# Autodesk Inventor assembly: A1-19037-200-00 30in lateral
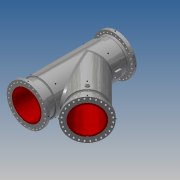
[picture p0: Inventor's stored thumbnail of the model, 180x180]
Saved by Autodesk Inventor 2017.3 (Build 213257000, 257)
## iProperties
Created: 2019-08-22
Part Number: A1-19037-200-00 30in lateral
Document SubType Name: Weldment
Designer: GVD
Project: A1-19037--CNUL Albian CST laterals
Weld Material: Steel, Mild, Welded
Mass: 6.1789e+06 g
Surface Area: 437297 cm^2
Volume: 814103 cm^3
Density: 7.58982 g/cm^3
Constructed By: Graeme_Van_Dongen
Project Name: CST laterals
Author: GVD
## Documents named in this file (15)
- C:\156Vault\A1 - Projects\A1-19\A1-19037--CNUL Albian CST laterals\A1-19037-200-00 30in lateral.iam
- N:\Inventor\Content Center Files\R2017\en-US\ANSI B18.3(08)\ANSI B18.3 - 1_2-13 UNC - 0.5(24).ipt
- N:\Inventor\Content Center Files\R2017\en-US\ASME B16.11(23)\ASME B16.11 Hex Head Plug 1_2.ipt
- N:\Inventor\Content Center Files\R2017\en-US\ASME B16.11(23)\ASME B16.11 Hex Head Plug 3_4.ipt
- N:\Inventor\Content Center Files\R2017\en-US\ASME B16.11(23)\ASME B16.11 Hex Head Plug 2.ipt
- C:\156Vault\A1 - Projects\A1-19\A1-19037--CNUL Albian CST laterals\A1-19037-200-04 30in CL300 RF flange - custom.ipt
- C:\156Vault\A1 - Projects\A1-19\A1-19037--CNUL Albian CST laterals\A1-19037-200-03 34in pipe.ipt
- C:\156Vault\A1 - Projects\A1-19\A1-19037--CNUL Albian CST laterals\A1-19037-200-01 Trunk shell.ipt
- C:\156Vault\A1 - Projects\A1-19\A1-19037--CNUL Albian CST laterals\A1-19037-200-02 Branch shell.ipt
- C:\156Vault\A1 - Projects\A1-19\A1-19037--CNUL Albian CST laterals\A1-19037-200-05 HCWI lateral.ipt
- C:\156Vault\A1 - Projects\A1-19\A1-19037--CNUL Albian CST laterals\A1-19037-200-06 HCWI liner - pup.ipt
- C:\156Vault\A1 - Projects\A1-19\A1-19037--CNUL Albian CST laterals\A1-19037-200-07 Trap rod.ipt
- C:\156Vault\A1 - Projects\A1-19\A1-19037--CNUL Albian CST laterals\A1-19037-200-08 2in x 38in threadolet.ipt
- C:\156Vault\A1 - Projects\Penticton Foundry\Tag mount - 6in.ipt
- C:\156Vault\A1 - Projects\A1-19\A1-19037--CNUL Albian CST laterals\A1-19037-200-03 34in pipe - flange assy.iam
## Components (61 placed, 14 different names)
1. A1-19037-200-04 30in CL300 RF flange - custom:2 — Insert:5, Insert:8, Mate:5, Angle:13, Angle:14, Mate:6, Mate:11, Angle:18, Mate:16, Angle:22, Tangent:5, Angle:23
2. A1-19037-200-04 30in CL300 RF flange - custom:3 — Insert:6, Insert:9, Mate:7, Angle:15, Angle:16, Mate:8, Mate:13, Angle:19, Mate:17, Angle:24, Tangent:6, Angle:25
3. A1-19037-200-05 HCWI lateral:1 — Insert:2, Angle:3, Insert:3, Angle:4, Insert:4, Angle:5, Flush:1, Mate:18, Angle:26
4. A1-19037-200-06 HCWI liner - pup:1 — Insert:2, Angle:3, Tangent:1
5. A1-19037-200-06 HCWI liner - pup:2 — Insert:3, Angle:4, Insert:5, Tangent:2
6. A1-19037-200-06 HCWI liner - pup:3 — Insert:4, Angle:5, Insert:6, Tangent:3
7. A1-19037-200-03 34in pipe:2 — Insert:8
8. A1-19037-200-03 34in pipe:3 — Insert:9
9. A1-19037-200-01 Trunk shell:1 — Flush:1, Mate:18, Angle:26, Flush:2, Mate:19, Angle:27, Mate:20, Angle:28, Tangent:7, Angle:29, Mate:21, Angle:30, Tangent:8, Angle:31, Mate:22, Angle:32, Tangent:9, Angle:33, Mate:23, Angle:34, Tangent:10, Angle:35, Tangent:12
10. A1-19037-200-02 Branch shell:1 — Flush:2, Mate:19, Angle:27, Mate:24, Mate:25, Angle:36, Mate:26, Angle:38, Tangent:11, Angle:39
11. ASME B16.11 Hex Head Plug 2:1 — Insert:10, Angle:37
12. A1-19037-200-08 2in x 38in threadolet:1 — Mate:24, Mate:25, Angle:36, Insert:10, Angle:37
13. A1-19037-200-03 34in pipe - flange assy:1 [sub-assembly]
14. A1-19037-200-07 Trap rod:1 — Tangent:1, Mate:10
15. Hexagon Socket Set Screw - Flat Point - Inch 1/2-13 UNC x 0.5:1 — Mate:10
16. ASME B16.11 Hex Head Plug 1/2:1
17. A1-19037-200-07 Trap rod:4
18. Hexagon Socket Set Screw - Flat Point - Inch 1/2-13 UNC x 0.5:4
19. ASME B16.11 Hex Head Plug 1/2:4
20. A1-19037-200-07 Trap rod:5
21. Hexagon Socket Set Screw - Flat Point - Inch 1/2-13 UNC x 0.5:5
22. ASME B16.11 Hex Head Plug 1/2:5
23. A1-19037-200-07 Trap rod:6
24. Hexagon Socket Set Screw - Flat Point - Inch 1/2-13 UNC x 0.5:6
25. ASME B16.11 Hex Head Plug 1/2:6
26. A1-19037-200-07 Trap rod:2 — Mate:5, Angle:13, Angle:14, Mate:6, Tangent:2, Mate:12
27. Hexagon Socket Set Screw - Flat Point - Inch 1/2-13 UNC x 0.5:2 — Mate:11, Mate:12, Angle:18
28. ASME B16.11 Hex Head Plug 1/2:2 — Mate:16, Angle:22, Tangent:5, Angle:23
29. A1-19037-200-07 Trap rod:7
30. Hexagon Socket Set Screw - Flat Point - Inch 1/2-13 UNC x 0.5:7
31. ASME B16.11 Hex Head Plug 1/2:7
32. A1-19037-200-07 Trap rod:8
33. Hexagon Socket Set Screw - Flat Point - Inch 1/2-13 UNC x 0.5:8
34. ASME B16.11 Hex Head Plug 1/2:8
35. A1-19037-200-07 Trap rod:9
36. Hexagon Socket Set Screw - Flat Point - Inch 1/2-13 UNC x 0.5:9
37. ASME B16.11 Hex Head Plug 1/2:9
38. A1-19037-200-07 Trap rod:3 — Mate:7, Angle:15, Angle:16, Mate:8, Tangent:3, Mate:14
39. Hexagon Socket Set Screw - Flat Point - Inch 1/2-13 UNC x 0.5:3 — Mate:13, Mate:14, Angle:19
40. ASME B16.11 Hex Head Plug 1/2:3 — Mate:17, Angle:24, Tangent:6, Angle:25
41. A1-19037-200-07 Trap rod:10
42. Hexagon Socket Set Screw - Flat Point - Inch 1/2-13 UNC x 0.5:10
43. ASME B16.11 Hex Head Plug 1/2:10
44. A1-19037-200-07 Trap rod:11
45. Hexagon Socket Set Screw - Flat Point - Inch 1/2-13 UNC x 0.5:11
46. ASME B16.11 Hex Head Plug 1/2:11
47. A1-19037-200-07 Trap rod:12
48. Hexagon Socket Set Screw - Flat Point - Inch 1/2-13 UNC x 0.5:12
49. ASME B16.11 Hex Head Plug 1/2:12
50. ASME B16.11 Hex Head Plug 3/4:1 — Mate:20, Angle:28, Tangent:7, Angle:29
51. ASME B16.11 Hex Head Plug 3/4:2 — Mate:21, Angle:30, Tangent:8, Angle:31
52. ASME B16.11 Hex Head Plug 3/4:3 — Mate:22, Angle:32, Tangent:9, Angle:33
53. ASME B16.11 Hex Head Plug 3/4:4 — Mate:23, Angle:34, Tangent:10, Angle:35
54. ASME B16.11 Hex Head Plug 3/4:5
55. ASME B16.11 Hex Head Plug 3/4:6
56. ASME B16.11 Hex Head Plug 3/4:7
57. ASME B16.11 Hex Head Plug 3/4:8
58. ASME B16.11 Hex Head Plug 3/4:9 — Mate:26, Angle:38, Tangent:11, Angle:39
59. ASME B16.11 Hex Head Plug 3/4:10
60. Tag mount - 6in:1 — Tangent:12
61. Tag mount - 6in:2
## Component patterns: (4 elements, first: A1-19037-200-07 Trap rod:1 + Hexagon Socket Set Screw - Flat Point - Inch 1/2-13 UNC x 0.5:1 + ASME B16.11 Hex Head Plug 1/2:1), (4 elements, first: A1-19037-200-07 Trap rod:2 + Hexagon Socket Set Screw - Flat Point - Inch 1/2-13 UNC x 0.5:2 + ASME B16.11 Hex Head Plug 1/2:2), (4 elements, first: A1-19037-200-07 Trap rod:3 + Hexagon Socket Set Screw - Flat Point - Inch 1/2-13 UNC x 0.5:3 + ASME B16.11 Hex Head Plug 1/2:3), (2 elements, first: ASME B16.11 Hex Head Plug 3/4:1 + ASME B16.11 Hex Head Plug 3/4:2 + ASME B16.11 Hex Head Plug 3/4:3 + ASME B16.11 Hex Head Plug 3/4:4), (2 elements, first: ASME B16.11 Hex Head Plug 3/4:9), (2 elements, first: Tag mount - 6in:1)
## Relationships (89: Angle 38, Mate 26, Tangent 12, Insert 9, Flush 4)
- [Mate]: A1-19037-200-03 34in pipe - flange assy:1
- [Mate]: A1-19037-200-03 34in pipe - flange assy:1
- [Angle] (0 deg): A1-19037-200-03 34in pipe - flange assy:1
- [Insert]: A1-19037-200-06 HCWI liner - pup:1 ↔ A1-19037-200-03 34in pipe - flange assy:1
- [Angle] (0 deg): A1-19037-200-06 HCWI liner - pup:1 ↔ A1-19037-200-03 34in pipe - flange assy:1
- Insert:2: A1-19037-200-05 HCWI lateral:1 ↔ A1-19037-200-06 HCWI liner - pup:1
- Angle:3 (0 deg): A1-19037-200-05 HCWI lateral:1 ↔ A1-19037-200-06 HCWI liner - pup:1
- Insert:3: A1-19037-200-05 HCWI lateral:1 ↔ A1-19037-200-06 HCWI liner - pup:2
- Angle:4 (0 deg): A1-19037-200-05 HCWI lateral:1 ↔ A1-19037-200-06 HCWI liner - pup:2
- Insert:4: A1-19037-200-05 HCWI lateral:1 ↔ A1-19037-200-06 HCWI liner - pup:3
- Angle:5 (0 deg): A1-19037-200-05 HCWI lateral:1 ↔ A1-19037-200-06 HCWI liner - pup:3
- Insert:5: A1-19037-200-04 30in CL300 RF flange - custom:2 ↔ A1-19037-200-06 HCWI liner - pup:2
- [Angle] (0 deg): A1-19037-200-04 30in CL300 RF flange - custom:2 ↔ A1-19037-200-03 34in pipe - flange assy:1
- Insert:6: A1-19037-200-04 30in CL300 RF flange - custom:3 ↔ A1-19037-200-06 HCWI liner - pup:3
- [Angle] (0 deg): A1-19037-200-04 30in CL300 RF flange - custom:3 ↔ A1-19037-200-03 34in pipe - flange assy:1
- Insert:8 (2.3813 mm): A1-19037-200-04 30in CL300 RF flange - custom:2 ↔ A1-19037-200-03 34in pipe:2
- [Angle] (0 deg): A1-19037-200-03 34in pipe:2 ↔ A1-19037-200-03 34in pipe - flange assy:1
- Insert:9 (2.3813 mm): A1-19037-200-04 30in CL300 RF flange - custom:3 ↔ A1-19037-200-03 34in pipe:3
- [Angle] (0 deg): A1-19037-200-03 34in pipe:3 ↔ A1-19037-200-03 34in pipe - flange assy:1
- [Mate]: A1-19037-200-03 34in pipe - flange assy:1 ↔ A1-19037-200-07 Trap rod:1
- [Angle] (0 deg): A1-19037-200-03 34in pipe - flange assy:1 ↔ A1-19037-200-07 Trap rod:1
- [Angle] (0 deg): A1-19037-200-03 34in pipe - flange assy:1 ↔ A1-19037-200-07 Trap rod:1
- [Mate] (0.3969 mm): A1-19037-200-03 34in pipe - flange assy:1 ↔ A1-19037-200-07 Trap rod:1
- Tangent:1: A1-19037-200-06 HCWI liner - pup:1 ↔ A1-19037-200-07 Trap rod:1
- Mate:5: A1-19037-200-04 30in CL300 RF flange - custom:2 ↔ A1-19037-200-07 Trap rod:2
- Angle:13 (0 deg): A1-19037-200-04 30in CL300 RF flange - custom:2 ↔ A1-19037-200-07 Trap rod:2
- Angle:14 (0 deg): A1-19037-200-04 30in CL300 RF flange - custom:2 ↔ A1-19037-200-07 Trap rod:2
- Mate:6 (0.3969 mm): A1-19037-200-04 30in CL300 RF flange - custom:2 ↔ A1-19037-200-07 Trap rod:2
- Tangent:2: A1-19037-200-06 HCWI liner - pup:2 ↔ A1-19037-200-07 Trap rod:2
- Mate:7: A1-19037-200-04 30in CL300 RF flange - custom:3 ↔ A1-19037-200-07 Trap rod:3
- Angle:15 (0 deg): A1-19037-200-04 30in CL300 RF flange - custom:3 ↔ A1-19037-200-07 Trap rod:3
- Angle:16 (0 deg): A1-19037-200-04 30in CL300 RF flange - custom:3 ↔ A1-19037-200-07 Trap rod:3
- Mate:8 (0.3969 mm): A1-19037-200-04 30in CL300 RF flange - custom:3 ↔ A1-19037-200-07 Trap rod:3
- Tangent:3: A1-19037-200-06 HCWI liner - pup:3 ↔ A1-19037-200-07 Trap rod:3
- [Mate]: A1-19037-200-03 34in pipe - flange assy:1 ↔ Hexagon Socket Set Screw - Flat Point - Inch 1/2-13 UNC x 0.5:1
- Mate:10: A1-19037-200-07 Trap rod:1 ↔ Hexagon Socket Set Screw - Flat Point - Inch 1/2-13 UNC x 0.5:1
- [Angle] (0 deg): A1-19037-200-03 34in pipe - flange assy:1 ↔ Hexagon Socket Set Screw - Flat Point - Inch 1/2-13 UNC x 0.5:1
- Mate:11: A1-19037-200-04 30in CL300 RF flange - custom:2 ↔ Hexagon Socket Set Screw - Flat Point - Inch 1/2-13 UNC x 0.5:2
- Mate:12: A1-19037-200-07 Trap rod:2 ↔ Hexagon Socket Set Screw - Flat Point - Inch 1/2-13 UNC x 0.5:2
- Angle:18 (0 deg): A1-19037-200-04 30in CL300 RF flange - custom:2 ↔ Hexagon Socket Set Screw - Flat Point - Inch 1/2-13 UNC x 0.5:2
- Mate:13: A1-19037-200-04 30in CL300 RF flange - custom:3 ↔ Hexagon Socket Set Screw - Flat Point - Inch 1/2-13 UNC x 0.5:3
- Mate:14: A1-19037-200-07 Trap rod:3 ↔ Hexagon Socket Set Screw - Flat Point - Inch 1/2-13 UNC x 0.5:3
- Angle:19 (0 deg): A1-19037-200-04 30in CL300 RF flange - custom:3 ↔ Hexagon Socket Set Screw - Flat Point - Inch 1/2-13 UNC x 0.5:3
- [Mate]: A1-19037-200-03 34in pipe - flange assy:1 ↔ ASME B16.11 Hex Head Plug 1/2:1
- [Angle] (180 deg): A1-19037-200-03 34in pipe - flange assy:1 ↔ ASME B16.11 Hex Head Plug 1/2:1
- [Tangent] (-11.7602 mm): A1-19037-200-03 34in pipe - flange assy:1 ↔ ASME B16.11 Hex Head Plug 1/2:1
- [Angle] (0 deg): A1-19037-200-03 34in pipe - flange assy:1 ↔ ASME B16.11 Hex Head Plug 1/2:1
- Mate:16: A1-19037-200-04 30in CL300 RF flange - custom:2 ↔ ASME B16.11 Hex Head Plug 1/2:2
- Angle:22 (180 deg): A1-19037-200-04 30in CL300 RF flange - custom:2 ↔ ASME B16.11 Hex Head Plug 1/2:2
- Tangent:5 (-11.7602 mm): A1-19037-200-04 30in CL300 RF flange - custom:2 ↔ ASME B16.11 Hex Head Plug 1/2:2
- Angle:23 (0 deg): A1-19037-200-04 30in CL300 RF flange - custom:2 ↔ ASME B16.11 Hex Head Plug 1/2:2
- Mate:17: A1-19037-200-04 30in CL300 RF flange - custom:3 ↔ ASME B16.11 Hex Head Plug 1/2:3
- Angle:24 (180 deg): A1-19037-200-04 30in CL300 RF flange - custom:3 ↔ ASME B16.11 Hex Head Plug 1/2:3
- Tangent:6 (-11.7602 mm): A1-19037-200-04 30in CL300 RF flange - custom:3 ↔ ASME B16.11 Hex Head Plug 1/2:3
- Angle:25 (0 deg): A1-19037-200-04 30in CL300 RF flange - custom:3 ↔ ASME B16.11 Hex Head Plug 1/2:3
- Flush:1: A1-19037-200-05 HCWI lateral:1 ↔ A1-19037-200-01 Trunk shell:1
- Mate:18: A1-19037-200-05 HCWI lateral:1 ↔ A1-19037-200-01 Trunk shell:1
- Angle:26 (0 deg): A1-19037-200-05 HCWI lateral:1 ↔ A1-19037-200-01 Trunk shell:1
- Flush:2: A1-19037-200-01 Trunk shell:1 ↔ A1-19037-200-02 Branch shell:1
- Mate:19: A1-19037-200-01 Trunk shell:1 ↔ A1-19037-200-02 Branch shell:1
- Angle:27 (45 deg): A1-19037-200-01 Trunk shell:1 ↔ A1-19037-200-02 Branch shell:1
- Mate:20: A1-19037-200-01 Trunk shell:1 ↔ ASME B16.11 Hex Head Plug 3/4:1
- Angle:28 (0 deg): A1-19037-200-01 Trunk shell:1 ↔ ASME B16.11 Hex Head Plug 3/4:1
- Tangent:7 (-12.2428 mm): A1-19037-200-01 Trunk shell:1 ↔ ASME B16.11 Hex Head Plug 3/4:1
- Angle:29 (0 deg): A1-19037-200-01 Trunk shell:1 ↔ ASME B16.11 Hex Head Plug 3/4:1
- Mate:21: A1-19037-200-01 Trunk shell:1 ↔ ASME B16.11 Hex Head Plug 3/4:2
- Angle:30 (180 deg): A1-19037-200-01 Trunk shell:1 ↔ ASME B16.11 Hex Head Plug 3/4:2
- Tangent:8 (-12.2428 mm): A1-19037-200-01 Trunk shell:1 ↔ ASME B16.11 Hex Head Plug 3/4:2
- Angle:31 (0 deg): A1-19037-200-01 Trunk shell:1 ↔ ASME B16.11 Hex Head Plug 3/4:2
- Mate:22: A1-19037-200-01 Trunk shell:1 ↔ ASME B16.11 Hex Head Plug 3/4:3
- Angle:32 (0 deg): A1-19037-200-01 Trunk shell:1 ↔ ASME B16.11 Hex Head Plug 3/4:3
- Tangent:9 (-12.2428 mm): A1-19037-200-01 Trunk shell:1 ↔ ASME B16.11 Hex Head Plug 3/4:3
- Angle:33 (0 deg): A1-19037-200-01 Trunk shell:1 ↔ ASME B16.11 Hex Head Plug 3/4:3
- Mate:23: A1-19037-200-01 Trunk shell:1 ↔ ASME B16.11 Hex Head Plug 3/4:4
- Angle:34 (180 deg): A1-19037-200-01 Trunk shell:1 ↔ ASME B16.11 Hex Head Plug 3/4:4
- Tangent:10 (-12.2428 mm): A1-19037-200-01 Trunk shell:1 ↔ ASME B16.11 Hex Head Plug 3/4:4
- Angle:35 (0 deg): A1-19037-200-01 Trunk shell:1 ↔ ASME B16.11 Hex Head Plug 3/4:4
- Mate:24: A1-19037-200-02 Branch shell:1 ↔ A1-19037-200-08 2in x 38in threadolet:1
- Mate:25: A1-19037-200-02 Branch shell:1 ↔ A1-19037-200-08 2in x 38in threadolet:1
- Angle:36 (0 deg): A1-19037-200-02 Branch shell:1 ↔ A1-19037-200-08 2in x 38in threadolet:1
- Insert:10 (-15.494 mm): ASME B16.11 Hex Head Plug 2:1 ↔ A1-19037-200-08 2in x 38in threadolet:1
- Angle:37 (0 deg): ASME B16.11 Hex Head Plug 2:1 ↔ A1-19037-200-08 2in x 38in threadolet:1
- Mate:26: A1-19037-200-02 Branch shell:1 ↔ ASME B16.11 Hex Head Plug 3/4:9
- Angle:38 (180 deg): A1-19037-200-02 Branch shell:1 ↔ ASME B16.11 Hex Head Plug 3/4:9
- Tangent:11 (-12.2428 mm): A1-19037-200-02 Branch shell:1 ↔ ASME B16.11 Hex Head Plug 3/4:9
- Angle:39 (0 deg): A1-19037-200-02 Branch shell:1 ↔ ASME B16.11 Hex Head Plug 3/4:9
- [Flush]: A1-19037-200-03 34in pipe - flange assy:1 ↔ Tag mount - 6in:1
- [Flush] (381 mm): A1-19037-200-03 34in pipe - flange assy:1 ↔ Tag mount - 6in:1
- Tangent:12: A1-19037-200-01 Trunk shell:1 ↔ Tag mount - 6in:1
